# Autodesk Inventor assembly: Assemblage_total_sur_toit
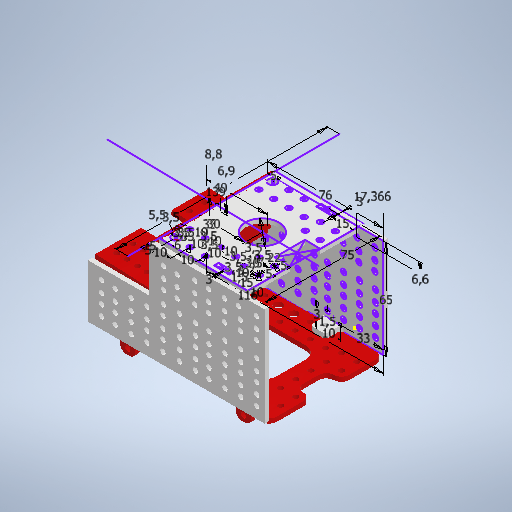
[picture p0: Inventor's stored thumbnail of the model, 512x512]
Saved by Autodesk Inventor 2025 (Build 290162000, 162)
## iProperties
Created: 2024-12-01
Part Number: Assemblage_total_sur_toit
Document SubType Name: Assembly
Designer: chass
Author: chass
## Documents named in this file (6)
- C:\Users\chass\Desktop\Extension_PAMI\Assemblage_total_sur_toit.iam
- C:\Users\chass\Desktop\Extension_PAMI\toit.ipt
- C:\Users\chass\Desktop\Extension_PAMI\mur_étage_droit.ipt
- C:\Users\chass\Desktop\Extension_PAMI\mur_étage_gauche.ipt
- C:\Users\chass\Desktop\Extension_PAMI\étage_servo.ipt
- C:\Users\chass\Desktop\Extension_PAMI\étage_BAU_et_étage_devant.iam
## Components (5 placed, 5 different names)
1. toit:1 — Placage:1, Placage:2, Placage:3, Placage:4, Placage:5, Placage:6
2. mur_étage_droit:1 — Placage:1, Placage:2, Placage:3
3. mur_étage_gauche:1 — Placage:4, Placage:5, Placage:6, Placage:8, Placage:9
4. étage_servo:1 — Placage:8
5. étage_BAU_et_étage_devant:1 [sub-assembly] — Placage:9
## Relationships (8: Mate 8)
- Placage:1 [Mate]: toit:1 ↔ mur_étage_droit:1
- Placage:2 [Mate]: toit:1 ↔ mur_étage_droit:1
- Placage:3 [Mate]: toit:1 ↔ mur_étage_droit:1
- Placage:4 [Mate]: toit:1 ↔ mur_étage_gauche:1
- Placage:5 [Mate]: toit:1 ↔ mur_étage_gauche:1
- Placage:6 [Mate]: toit:1 ↔ mur_étage_gauche:1
- Placage:8 [Mate]: mur_étage_gauche:1 ↔ étage_servo:1
- Placage:9 [Mate]: mur_étage_gauche:1 ↔ étage_BAU_et_étage_devant:1
